# Autodesk Inventor assembly: Stop Button
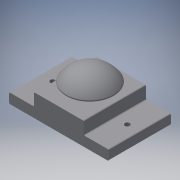
[picture p0: Inventor's stored thumbnail of the model, 180x180]
Saved by Autodesk Inventor 2019 (Build 230136000, 136)
## iProperties
Created: 2019-02-14
Part Number: Stop Button
Document SubType Name: Assembly
Designer: lopez.xavier
Author: lopez.xavier
## Documents named in this file (3)
- \\fs1\studentusers\class19\Lopez.Xavier\documents\Cad\Dr. Julius Strange Pork\Stop Button\Stop Button.iam
- \\fs1\studentusers\class19\Lopez.Xavier\documents\Cad\Dr. Julius Strange Pork\Stop Button\Base.ipt
- \\fs1\studentusers\class19\Lopez.Xavier\documents\Cad\Dr. Julius Strange Pork\Stop Button\Button.ipt
## Components (2 placed, 2 different names)
1. Base:1 — Mate:1, Mate:2, Mate:3
2. Button:1 — Mate:1, Mate:2, Mate:3
## Relationships (3: Mate 3)
- Mate:1: Base:1 ↔ Button:1
- Mate:2: Base:1 ↔ Button:1
- Mate:3 (2.54 mm): Base:1 ↔ Button:1
